# Autodesk Inventor assembly: A2017_T5_05
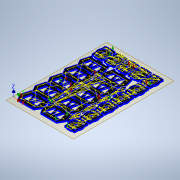
[picture p0: Inventor's stored thumbnail of the model, 180x180]
Saved by Autodesk Inventor 2022 (Build 260153000, 153)
## iProperties
Created: 2022-09-28
Part Number: A2017_T5_05
Document SubType Name: Assembly
Designer: Masato
Author: Masato
## Documents named in this file (5)
- C:\Users\6343y\ドキュメント\Inventor\SUSTAINA-OP\Cam\A2017_T5\A2017_T5_05.iam
- C:\Users\6343y\ドキュメント\Inventor\SUSTAINA-OP\Cam\DisposableBoard.ipt
- C:\Users\6343y\ドキュメント\Inventor\SUSTAINA-OP\UpperBody\Trunk\Trunk_lower_side_frame.ipt
- C:\Users\6343y\ドキュメント\Inventor\SUSTAINA-OP\LowerBody\Foot\Foot_root_block.ipt
- C:\Users\6343y\ドキュメント\Inventor\SUSTAINA-OP\UpperBody\UpperBody_horn_frame.ipt
## Components (33 placed, 4 different names)
1. DisposableBoard:1 — フラッシュ:1, フラッシュ:2, フラッシュ:3, フラッシュ:4, フラッシュ:5, 正接:1, フラッシュ:6, 正接:2, フラッシュ:7, 正接:3
2. Trunk_lower_side_frame:1 — メイト:1, フラッシュ:5, 正接:1
3. Trunk_lower_side_frame:2 — メイト:7
4. Trunk_lower_side_frame:3
5. Trunk_lower_side_frame:4
6. Trunk_lower_side_frame:5
7. Trunk_lower_side_frame:6 — メイト:9, メイト:12
8. Trunk_lower_side_frame:7 — メイト:8, メイト:15
9. Trunk_lower_side_frame:8
10. Trunk_lower_side_frame:9
11. Trunk_lower_side_frame:10
12. UpperBody_horn_frame:1 — メイト:6, フラッシュ:6, 正接:2
13. UpperBody_horn_frame:3
14. UpperBody_horn_frame:4
15. UpperBody_horn_frame:5
16. UpperBody_horn_frame:6
17. UpperBody_horn_frame:2 — メイト:10, フラッシュ:7, 正接:3
18. UpperBody_horn_frame:7
19. UpperBody_horn_frame:8
20. UpperBody_horn_frame:9
21. UpperBody_horn_frame:10
22. Foot_root_block:1 — メイト:2, メイト:7, メイト:8, メイト:9
23. Foot_root_block:2
24. Foot_root_block:3
25. Foot_root_block:4
26. Foot_root_block:5 — メイト:11, メイト:12, メイト:14
27. Foot_root_block:6 — メイト:13, メイト:14, メイト:15
28. Foot_root_block:7
29. Foot_root_block:8
30. Foot_root_block:9
31. Foot_root_block:10
32. Foot_root_block:11
33. Foot_root_block:12
## Component patterns: (10 elements, first: Trunk_lower_side_frame:1), (5 elements, first: UpperBody_horn_frame:1), (5 elements, first: UpperBody_horn_frame:2), (4 elements, first: Foot_root_block:1), (4 elements, first: Foot_root_block:5 + Foot_root_block:6)
## Relationships (22: Mate 12, Flush 7, Tangent 3)
- フラッシュ:1 [Flush]: DisposableBoard:1
- フラッシュ:2 [Flush]: DisposableBoard:1
- フラッシュ:3 [Flush]: DisposableBoard:1
- フラッシュ:4 [Flush]: DisposableBoard:1
- メイト:1 [Mate]: Trunk_lower_side_frame:1
- フラッシュ:5 [Flush] (2.1 mm): DisposableBoard:1 ↔ Trunk_lower_side_frame:1
- 正接:1 [Tangent] (2.1 mm): DisposableBoard:1 ↔ Trunk_lower_side_frame:1
- メイト:2 [Mate]: Foot_root_block:1
- メイト:6 [Mate]: UpperBody_horn_frame:1
- メイト:7 [Mate] (2.1 mm): Trunk_lower_side_frame:2 ↔ Foot_root_block:1
- メイト:8 [Mate] (2.1 mm): Trunk_lower_side_frame:7 ↔ Foot_root_block:1
- メイト:9 [Mate] (2.1 mm): Trunk_lower_side_frame:6 ↔ Foot_root_block:1
- フラッシュ:6 [Flush] (2.1 mm): DisposableBoard:1 ↔ UpperBody_horn_frame:1
- 正接:2 [Tangent] (2.1 mm): DisposableBoard:1 ↔ UpperBody_horn_frame:1
- メイト:10 [Mate]: UpperBody_horn_frame:2
- フラッシュ:7 [Flush] (2.1 mm): DisposableBoard:1 ↔ UpperBody_horn_frame:2
- 正接:3 [Tangent] (2.1 mm): DisposableBoard:1 ↔ UpperBody_horn_frame:2
- メイト:11 [Mate]: Foot_root_block:5
- メイト:12 [Mate] (2.1 mm): Trunk_lower_side_frame:6 ↔ Foot_root_block:5
- メイト:13 [Mate]: Foot_root_block:6
- メイト:14 [Mate] (2.1 mm): Foot_root_block:5 ↔ Foot_root_block:6
- メイト:15 [Mate] (2.1 mm): Trunk_lower_side_frame:7 ↔ Foot_root_block:6
